# Autodesk Inventor assembly: original_flatcov_5mm
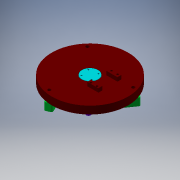
[picture p0: Inventor's stored thumbnail of the model, 180x180]
Saved by Autodesk Inventor 2018 (Build 220112000, 112)
## iProperties
Created: 2019-01-24
Part Number: original_flatcov_5mm
Material: 一般
Document SubType Name: Assembly
Designer: lowyu
Author: lowyu
## Documents named in this file (5)
- C:\Users\lowyu\Desktop\HAND\シャッターハンド\卒論\originals\original_flatcov_5mm.iam
- C:\Users\lowyu\Desktop\HAND\シャッターハンド\卒論\originals\parts\rotate_plate_4.ipt
- C:\Users\lowyu\Desktop\HAND\シャッターハンド\卒論\originals\parts\fix_plate_3.ipt
- C:\Users\lowyu\Desktop\HAND\シャッターハンド\卒論\originals\parts\finger_4_5mm.ipt
- C:\Users\lowyu\Desktop\HAND\シャッターハンド\卒論\originals\parts\flat_cover_5mm.ipt
## Components (8 placed, 4 different names)
1. rotate_plate_4:1 — メイト:3, メイト:4, メイト:5, メイト:6
2. fix_plate_3:1 — メイト:3, メイト:4
3. finger_4_5mm:1 — メイト:1, メイト:2, メイト:5, メイト:6
4. flat_cover_5mm:1 — メイト:1, メイト:2
5. finger_4_5mm:2
6. flat_cover_5mm:2
7. finger_4_5mm:3
8. flat_cover_5mm:3
## Component patterns: (3 elements, first: finger_4_5mm:1 + flat_cover_5mm:1)
## Relationships (6: Mate 6)
- メイト:1 [Mate]: finger_4_5mm:1 ↔ flat_cover_5mm:1
- メイト:2 [Mate]: finger_4_5mm:1 ↔ flat_cover_5mm:1
- メイト:3 [Mate]: rotate_plate_4:1 ↔ fix_plate_3:1
- メイト:4 [Mate]: rotate_plate_4:1 ↔ fix_plate_3:1
- メイト:5 [Mate]: rotate_plate_4:1 ↔ finger_4_5mm:1
- メイト:6 [Mate]: rotate_plate_4:1 ↔ finger_4_5mm:1
